# Autodesk Inventor assembly: zlozenie
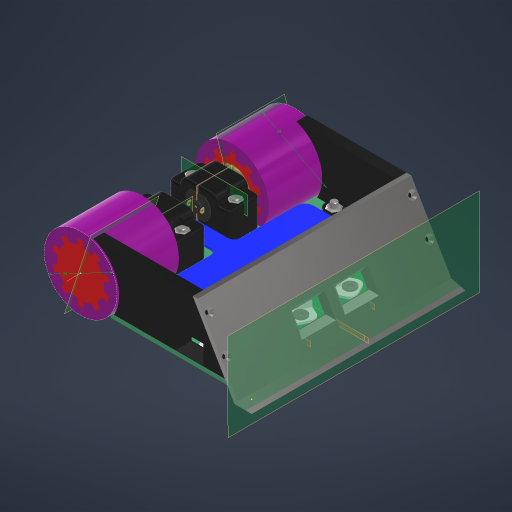
[picture p0: Inventor's stored thumbnail of the model, 512x512]
Saved by Autodesk Inventor 2024 (Build 280153000, 153)
## iProperties
Created: 2024-05-23
Part Number: zlozenie
Document SubType Name: Assembly
Designer: Adam
Mass: 228.786 g
Surface Area: 710.183 cm^2
Volume: 83.5462 cm^3
Density: 2.73844 g/cm^3
Author: Adam
## Documents named in this file (25)
- C:\Users\pryst\Desktop\KoNaR\Warsztaty\minisumo\model\zlozenie.iam
- C:\Users\pryst\Desktop\KoNaR\Warsztaty\minisumo\model\czujnik_odbibiowy.ipt
- C:\Users\pryst\Desktop\KoNaR\Warsztaty\minisumo\model\modele_stp\modele_stp\N20 DC MOTOR\N20 DC MOTOR.ipt
- C:\Users\pryst\Desktop\KoNaR\Warsztaty\minisumo\model\modele_stp\modele_stp\TOF VL53L0X\TOF VL53L0X.ipt
- C:\Users\pryst\Desktop\KoNaR\Warsztaty\minisumo\model\felga.ipt
- C:\Users\pryst\Desktop\KoNaR\Warsztaty\minisumo\model\podstawa.ipt
- C:\Users\pryst\Desktop\KoNaR\Warsztaty\minisumo\model\mocowanie_silnika.ipt
- C:\Users\pryst\Desktop\KoNaR\Warsztaty\minisumo\model\podstawka silnika.ipt
- C:\Users\pryst\Desktop\KoNaR\Warsztaty\minisumo\model\opona.ipt
- C:\Users\pryst\Desktop\KoNaR\Warsztaty\minisumo\model\lemiesz.ipt
- C:\Users\pryst\Desktop\KoNaR\Warsztaty\minisumo\model\modele_stp\modele_stp\N20 DC MOTOR\N20 DC MOTOR_CPY.ipt
- C:\Users\pryst\Desktop\KoNaR\Warsztaty\minisumo\model\mocowanie_silnika_CPY.ipt
- C:\Users\pryst\Desktop\KoNaR\Warsztaty\minisumo\model\podstawka silnika_CPY.ipt
- C:\Users\pryst\Desktop\KoNaR\Warsztaty\minisumo\model\mocowanie_tofa.ipt
- C:\Users\pryst\Desktop\KoNaR\Warsztaty\minisumo\model\modele_stp\modele_stp\TOF VL53L0X\TOF VL53L0X_CPY.ipt
- C:\Users\pryst\Desktop\KoNaR\Warsztaty\minisumo\model\modele_stp\modele_stp\TOF VL53L0X\TOF VL53L0X_CPY1.ipt
- C:\Users\pryst\Desktop\KoNaR\Warsztaty\minisumo\model\modele_stp\modele_stp\TOF VL53L0X\TOF VL53L0X_CPY_CPY.ipt
- C:\Users\pryst\Desktop\KoNaR\Warsztaty\minisumo\model\bok_lewy.ipt
- C:\Users\pryst\Desktop\KoNaR\Warsztaty\minisumo\model\bok_prawy.ipt
- C:\Users\pryst\Desktop\KoNaR\Warsztaty\minisumo\model\pcb.ipt
- C:\Users\pryst\Desktop\KoNaR\Warsztaty\minisumo\model\podkladka.ipt
- C:\Users\pryst\Documents\Inventor\Content Center Files\R2024\en-US\DIN 934\DIN 934 - M3 x 0,5.ipt
- C:\Users\pryst\Documents\Inventor\Content Center Files\R2024\en-US\DIN 7991(1)\DIN 7991 - M3  x  8.ipt
- C:\Users\pryst\Documents\Inventor\Content Center Files\R2024\en-US\ANSI B18.3.4M(2)\ANSI B18.3.4M - M3 x 0.5 x 10(1).ipt
- C:\Users\pryst\Documents\Inventor\Content Center Files\R2024\en-US\DIN 7991(1)\DIN 7991 - M3  x  16.ipt
## Components (55 placed, 24 different names)
1. czujnik_odbibiowy:1 — Mate:28
2. N20 DC MOTOR:1 — Insert:1, Mate:5, Mate:6
3. TOF VL53L0X:1 — Mate:20, Insert:12
4. felga:1 — Insert:1, Insert:3
5. podstawa:1 — Flush:2, Mate:9, Flush:8, Mate:13, Flush:9, Mate:14, Flush:12, Mate:18, Mate:20, Angle:1, Flush:14, Mate:22, Mate:23, Mate:24, Angle:2, Angle:3, Mate:25, Flush:18, Flush:19, Flush:20, Mate:26, Flush:21, Flush:22, Mate:27, Insert:20, Insert:21, Insert:28, Insert:29, Insert:31, Insert:32, Insert:33, Insert:34, Insert:35, Mate:32, Mate:33, Mate:40, Mate:41, Mate:42, Mate:43
6. mocowanie_silnika:1 — Mate:8, Flush:4, Flush:5, Insert:22, Insert:23
7. podstawka silnika:1 — Flush:2, Mate:5, Mate:6, Mate:8, Flush:4, Mate:9, Flush:5, Mate:14, Flush:13
8. opona:1 — Insert:3
9. lemiesz:1 — Mate:13, Flush:9, Flush:14, Flush:16
10. N20 DC MOTOR_CPY:1 — Mate:16, Mate:17, Mate:19, Insert:11
11. mocowanie_silnika_CPY:1 — Flush:10, Flush:11, Mate:15, Insert:24, Insert:25
12. podstawka silnika_CPY:1 — Flush:10, Flush:11, Mate:15, Mate:16, Mate:17, Flush:12, Mate:18, Flush:13, Mate:19
13. mocowanie_tofa:1 — Angle:1, Insert:12, Insert:21, Mate:45
14. TOF VL53L0X_CPY:1 — Insert:14
15. TOF VL53L0X_CPY1:1 — Insert:13
16. TOF VL53L0X_CPY_CPY:1 — Insert:15, Flush:24
17. felga:2 — Insert:10, Insert:11
18. opona:2 — Insert:10
19. mocowanie_tofa:2 — Mate:22, Insert:13, Insert:20, Mate:46
20. mocowanie_tofa:3 — Mate:23, Insert:14, Angle:3, Mate:44
21. mocowanie_tofa:4 — Mate:24, Insert:15, Angle:2, Mate:47
22. bok_lewy:1 — Mate:25, Flush:18, Flush:19, Insert:27
23. bok_prawy:1 — Flush:20, Mate:26, Flush:21, Insert:26
24. pcb:1 — Insert:16, Insert:17, Insert:18, Mate:28, Mate:29, Mate:30, Mate:34, Mate:35, Mate:36, Mate:37, Mate:38, Mate:39
25. podkladka:1 — Insert:16, Mate:27
26. podkladka:2 — Insert:17
27. podkladka:3 — Insert:18
28. czujnik_odbibiowy:3 — Mate:30
29. czujnik_odbibiowy:4 — Mate:29
30. DIN 934 - replaced by DIN EN 24032/28673/28674 M3:1 — Insert:22
31. DIN 934 - replaced by DIN EN 24032/28673/28674 M3:2 — Insert:23
32. DIN 934 - replaced by DIN EN 24032/28673/28674 M3:3 — Insert:24
33. DIN 934 - replaced by DIN EN 24032/28673/28674 M3:4 — Insert:25
34. DIN 934 - replaced by DIN EN 24032/28673/28674 M3:5 — Insert:26
35. DIN 934 - replaced by DIN EN 24032/28673/28674 M3:6 — Insert:27
36. DIN 934 - replaced by DIN EN 24032/28673/28674 M3:7 — Insert:28
37. DIN 934 - replaced by DIN EN 24032/28673/28674 M3:8 — Insert:29
38. DIN 934 - replaced by DIN EN 24032/28673/28674 M3:10 — Insert:31
39. DIN 934 - replaced by DIN EN 24032/28673/28674 M3:11 — Insert:32
40. DIN 934 - replaced by DIN EN 24032/28673/28674 M3:12 — Insert:33
41. DIN 934 - replaced by DIN EN 24032/28673/28674 M3:13 — Insert:34
42. DIN 934 - replaced by DIN EN 24032/28673/28674 M3:14 — Insert:35
43. DIN 7991 - replaced by DIN EN ISO 10642 M3  x  8:2 — Mate:32
44. DIN 7991 - replaced by DIN EN ISO 10642 M3  x  8:3 — Mate:33
45. Forged Hexagon Socket Button Head Cap Screw - Metric M3 x 0.5 x 10:1 — Mate:34, Mate:35
46. Forged Hexagon Socket Button Head Cap Screw - Metric M3 x 0.5 x 10:2 — Mate:36, Mate:37
47. Forged Hexagon Socket Button Head Cap Screw - Metric M3 x 0.5 x 10:3 — Mate:38, Mate:39
48. DIN 7991 - replaced by DIN EN ISO 10642 M3  x  16:1 — Mate:40
49. DIN 7991 - replaced by DIN EN ISO 10642 M3  x  16:2 — Mate:41
50. DIN 7991 - replaced by DIN EN ISO 10642 M3  x  16:3 — Mate:43
51. DIN 7991 - replaced by DIN EN ISO 10642 M3  x  16:4 — Mate:42
52. DIN 7991 - replaced by DIN EN ISO 10642 M3  x  8:4 — Mate:44
53. DIN 7991 - replaced by DIN EN ISO 10642 M3  x  8:5 — Mate:45
54. DIN 7991 - replaced by DIN EN ISO 10642 M3  x  8:6 — Mate:46
55. DIN 7991 - replaced by DIN EN ISO 10642 M3  x  8:7 — Mate:47
## Relationships (84: Mate 37, Insert 26, Flush 18, Angle 3)
- Insert:1: N20 DC MOTOR:1 ↔ felga:1
- Flush:2: podstawa:1 ↔ podstawka silnika:1
- Mate:5: N20 DC MOTOR:1 ↔ podstawka silnika:1
- Mate:6: N20 DC MOTOR:1 ↔ podstawka silnika:1
- Mate:8: mocowanie_silnika:1 ↔ podstawka silnika:1
- Flush:4: mocowanie_silnika:1 ↔ podstawka silnika:1
- Mate:9: podstawa:1 ↔ podstawka silnika:1
- Flush:5: mocowanie_silnika:1 ↔ podstawka silnika:1
- Insert:3: felga:1 ↔ opona:1
- Flush:8: podstawa:1
- Mate:13: podstawa:1 ↔ lemiesz:1
- Flush:9: podstawa:1 ↔ lemiesz:1
- Mate:14: podstawa:1 ↔ podstawka silnika:1
- Flush:10: mocowanie_silnika_CPY:1 ↔ podstawka silnika_CPY:1
- Flush:11: mocowanie_silnika_CPY:1 ↔ podstawka silnika_CPY:1
- Mate:15: mocowanie_silnika_CPY:1 ↔ podstawka silnika_CPY:1
- Mate:16: N20 DC MOTOR_CPY:1 ↔ podstawka silnika_CPY:1
- Mate:17: N20 DC MOTOR_CPY:1 ↔ podstawka silnika_CPY:1
- Flush:12: podstawa:1 ↔ podstawka silnika_CPY:1
- Mate:18: podstawa:1 ↔ podstawka silnika_CPY:1
- Flush:13: podstawka silnika:1 ↔ podstawka silnika_CPY:1
- Mate:19: N20 DC MOTOR_CPY:1 ↔ podstawka silnika_CPY:1
- Mate:20: TOF VL53L0X:1 ↔ podstawa:1
- Angle:1 (25 deg): podstawa:1 ↔ mocowanie_tofa:1
- Flush:14 (6 mm): podstawa:1 ↔ lemiesz:1
- Insert:10: felga:2 ↔ opona:2
- Insert:11: N20 DC MOTOR_CPY:1 ↔ felga:2
- Flush:16: lemiesz:1
- Insert:12: TOF VL53L0X:1 ↔ mocowanie_tofa:1
- Mate:22: podstawa:1 ↔ mocowanie_tofa:2
- Mate:23: podstawa:1 ↔ mocowanie_tofa:3
- Mate:24: podstawa:1 ↔ mocowanie_tofa:4
- Insert:13: TOF VL53L0X_CPY1:1 ↔ mocowanie_tofa:2
- Insert:14: TOF VL53L0X_CPY:1 ↔ mocowanie_tofa:3
- Insert:15: TOF VL53L0X_CPY_CPY:1 ↔ mocowanie_tofa:4
- Angle:2 (-90 deg): podstawa:1 ↔ mocowanie_tofa:4
- Angle:3 (90 deg): podstawa:1 ↔ mocowanie_tofa:3
- Mate:25: podstawa:1 ↔ bok_lewy:1
- Flush:18: podstawa:1 ↔ bok_lewy:1
- Flush:19: podstawa:1 ↔ bok_lewy:1
- Flush:20: podstawa:1 ↔ bok_prawy:1
- Mate:26: podstawa:1 ↔ bok_prawy:1
- Flush:21: podstawa:1 ↔ bok_prawy:1
- Flush:22 (15 mm): podstawa:1
- Flush:23 (-30 mm)
- Insert:16: pcb:1 ↔ podkladka:1
- Insert:17: pcb:1 ↔ podkladka:2
- Insert:18: pcb:1 ↔ podkladka:3
- Mate:27: podstawa:1 ↔ podkladka:1
- Insert:20: podstawa:1 ↔ mocowanie_tofa:2
- Insert:21: podstawa:1 ↔ mocowanie_tofa:1
- Mate:28: czujnik_odbibiowy:1 ↔ pcb:1
- Mate:29: pcb:1 ↔ czujnik_odbibiowy:4
- Mate:30: pcb:1 ↔ czujnik_odbibiowy:3
- Flush:24 (-30 mm): TOF VL53L0X_CPY_CPY:1
- Insert:22: mocowanie_silnika:1 ↔ DIN 934 - replaced by DIN EN 24032/28673/28674 M3:1
- Insert:23: mocowanie_silnika:1 ↔ DIN 934 - replaced by DIN EN 24032/28673/28674 M3:2
- Insert:24: mocowanie_silnika_CPY:1 ↔ DIN 934 - replaced by DIN EN 24032/28673/28674 M3:3
- Insert:25: mocowanie_silnika_CPY:1 ↔ DIN 934 - replaced by DIN EN 24032/28673/28674 M3:4
- Insert:26: bok_prawy:1 ↔ DIN 934 - replaced by DIN EN 24032/28673/28674 M3:5
- Insert:27: bok_lewy:1 ↔ DIN 934 - replaced by DIN EN 24032/28673/28674 M3:6
- Insert:28: podstawa:1 ↔ DIN 934 - replaced by DIN EN 24032/28673/28674 M3:7
- Insert:29: podstawa:1 ↔ DIN 934 - replaced by DIN EN 24032/28673/28674 M3:8
- Insert:31: podstawa:1 ↔ DIN 934 - replaced by DIN EN 24032/28673/28674 M3:10
- Insert:32: podstawa:1 ↔ DIN 934 - replaced by DIN EN 24032/28673/28674 M3:11
- Insert:33: podstawa:1 ↔ DIN 934 - replaced by DIN EN 24032/28673/28674 M3:12
- Insert:34: podstawa:1 ↔ DIN 934 - replaced by DIN EN 24032/28673/28674 M3:13
- Insert:35: podstawa:1 ↔ DIN 934 - replaced by DIN EN 24032/28673/28674 M3:14
- Mate:32: podstawa:1 ↔ DIN 7991 - replaced by DIN EN ISO 10642 M3  x  8:2
- Mate:33: podstawa:1 ↔ DIN 7991 - replaced by DIN EN ISO 10642 M3  x  8:3
- Mate:34: pcb:1 ↔ Forged Hexagon Socket Button Head Cap Screw - Metric M3 x 0.5 x 10:1
- Mate:35: pcb:1 ↔ Forged Hexagon Socket Button Head Cap Screw - Metric M3 x 0.5 x 10:1
- Mate:36: pcb:1 ↔ Forged Hexagon Socket Button Head Cap Screw - Metric M3 x 0.5 x 10:2
- Mate:37: pcb:1 ↔ Forged Hexagon Socket Button Head Cap Screw - Metric M3 x 0.5 x 10:2
- Mate:38: pcb:1 ↔ Forged Hexagon Socket Button Head Cap Screw - Metric M3 x 0.5 x 10:3
- Mate:39: pcb:1 ↔ Forged Hexagon Socket Button Head Cap Screw - Metric M3 x 0.5 x 10:3
- Mate:40: podstawa:1 ↔ DIN 7991 - replaced by DIN EN ISO 10642 M3  x  16:1
- Mate:41: podstawa:1 ↔ DIN 7991 - replaced by DIN EN ISO 10642 M3  x  16:2
- Mate:42: podstawa:1 ↔ DIN 7991 - replaced by DIN EN ISO 10642 M3  x  16:4
- Mate:43: podstawa:1 ↔ DIN 7991 - replaced by DIN EN ISO 10642 M3  x  16:3
- Mate:44: mocowanie_tofa:3 ↔ DIN 7991 - replaced by DIN EN ISO 10642 M3  x  8:4
- Mate:45: mocowanie_tofa:1 ↔ DIN 7991 - replaced by DIN EN ISO 10642 M3  x  8:5
- Mate:46: mocowanie_tofa:2 ↔ DIN 7991 - replaced by DIN EN ISO 10642 M3  x  8:6
- Mate:47: mocowanie_tofa:4 ↔ DIN 7991 - replaced by DIN EN ISO 10642 M3  x  8:7
